# Autodesk Inventor assembly: main
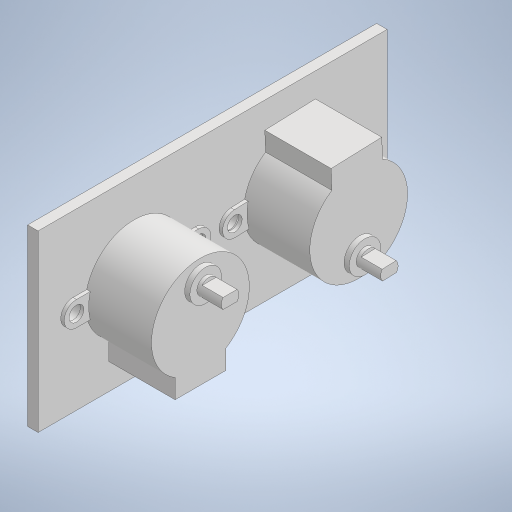
[picture p0: Inventor's stored thumbnail of the model, 512x512]
Saved by Autodesk Inventor 2023 (Build 270158000, 158)
## iProperties
Created: 2022-04-18
Part Number: main
Document SubType Name: Assembly
Designer: carson
Author: carson
## Documents named in this file (5)
- C:\Users\carson\Desktop\cad\whiteboard\main.iam
- C:\Users\carson\Desktop\cad\whiteboard\board.ipt
- C:\Users\carson\Desktop\cad\whiteboard\marker.ipt
- C:\Users\carson\Desktop\cad\whiteboard\motor.ipt
- C:\Users\carson\Desktop\cad\whiteboard\motorPlate.ipt
## Components (5 placed, 4 different names)
1. board:1 — Mate:1
2. marker:1 — Mate:1
3. motor:1 — Mate:5
4. motor:2 — Mate:2, Mate:3, Mate:4
5. motorPlate:1 — Mate:2, Mate:3, Mate:4, Mate:5
## Relationships (5: Mate 5)
- Mate:1: board:1 ↔ marker:1
- Mate:2: motor:2 ↔ motorPlate:1
- Mate:3: motor:2 ↔ motorPlate:1
- Mate:4: motor:2 ↔ motorPlate:1
- Mate:5: motor:1 ↔ motorPlate:1
